# Autodesk Inventor assembly: Small Wheel
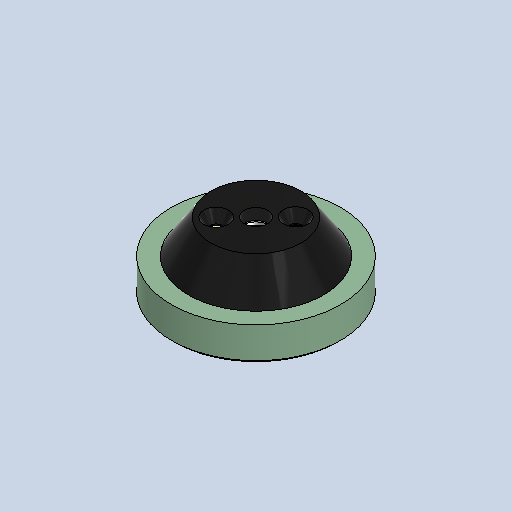
[picture p0: Inventor's stored thumbnail of the model, 512x512]
Saved by Autodesk Inventor 2023.4 (Build 274418000, 418)
## iProperties
Created: 2024-05-15
Part Number: Small Wheel
Document SubType Name: Assembly
Designer: Nathan Cai
Author: Nathan Cai
## Documents named in this file (4)
- E:\Documents\Inventor\Law - V2.1\Pusher Module - Law\Small Wheel.iam
- E:\Documents\Inventor\Law - V2.1\Pusher Module - Law\Hub Adapter.ipt
- E:\Documents\Inventor\Law - V2.1\Pusher Module - Law\Hubs - 6mm.ipt
- E:\Documents\Inventor\Law - V2.1\Pusher Module - Law\Custom Wheel V1.0\Recessed Wheels V1.0.iam
## Components (3 placed, 3 different names)
1. Hub Adapter:1 — Mate:1, Mate:2, Mate:4
2. Hubs - 6mm:1 — Mate:1, Mate:2, Mate:3
3. Recessed Wheels V1.0:1 [sub-assembly] — Mate:3, Mate:4
## Relationships (4: Mate 4)
- Mate:1: Hub Adapter:1 ↔ Hubs - 6mm:1
- Mate:2: Hub Adapter:1 ↔ Hubs - 6mm:1
- Mate:3: Hubs - 6mm:1 ↔ Recessed Wheels V1.0:1
- Mate:4: Hub Adapter:1 ↔ Recessed Wheels V1.0:1
